# Autodesk Inventor assembly: Z Axis Motor Mount
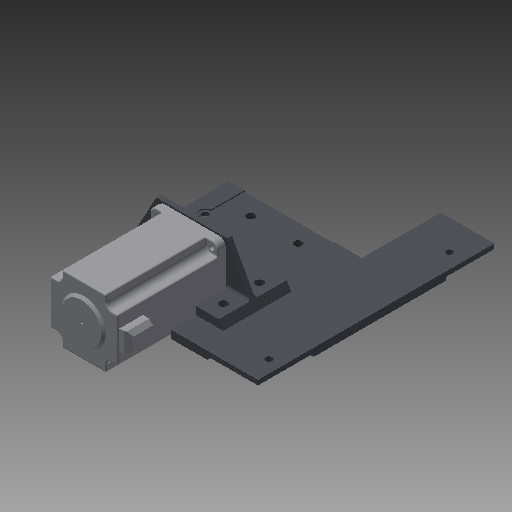
[picture p0: Inventor's stored thumbnail of the model, 512x512]
Saved by Autodesk Inventor 2018 (Build 220112000, 112)
## iProperties
Created: 2018-04-10
Part Number: Z Axis Motor Mount
Document SubType Name: Assembly
Designer: M224826
Author: M224826
## Documents named in this file (4)
- C:\Users\M224826\Documents\GitHub\CNC-Lathe-CAD\CNC Lathe Project\Project Files\Z Axis Motor Mount\Z Axis Motor Mount.iam
- C:\Users\M224826\Documents\GitHub\CNC-Lathe-CAD\CNC Lathe Project\Project Files\Servo Motor\Servo Motor.iam
- C:\Users\M224826\Documents\GitHub\CNC-Lathe-CAD\CNC Lathe Project\Project Files\Z Axis Motor Mount\Motor Support Fin.ipt
- C:\Users\M224826\Documents\GitHub\CNC-Lathe-CAD\CNC Lathe Project\Project Files\Z Axis Motor Mount\SUPPORT MAIN FRAME MOTOR-BALL SCREW-REV-B.ipt
## Components (3 placed, 3 different names)
1. Servo Motor:1 [sub-assembly] — Mate:5, Mate:6, Mate:7
2. Motor Support Fin:1 — Mate:2, Mate:3, Mate:4, Mate:5, Mate:6, Mate:7
3. SUPPORT MAIN FRAME MOTOR-BALL SCREW-REV-B:1 — Mate:1, Flush:1, Flush:2, Mate:2, Mate:3, Mate:4
## Relationships (9: Mate 7, Flush 2)
- Mate:1: SUPPORT MAIN FRAME MOTOR-BALL SCREW-REV-B:1
- Flush:1: SUPPORT MAIN FRAME MOTOR-BALL SCREW-REV-B:1
- Flush:2: SUPPORT MAIN FRAME MOTOR-BALL SCREW-REV-B:1
- Mate:2: Motor Support Fin:1 ↔ SUPPORT MAIN FRAME MOTOR-BALL SCREW-REV-B:1
- Mate:3: Motor Support Fin:1 ↔ SUPPORT MAIN FRAME MOTOR-BALL SCREW-REV-B:1
- Mate:4: Motor Support Fin:1 ↔ SUPPORT MAIN FRAME MOTOR-BALL SCREW-REV-B:1
- Mate:5: Servo Motor:1 ↔ Motor Support Fin:1
- Mate:6: Servo Motor:1 ↔ Motor Support Fin:1
- Mate:7: Servo Motor:1 ↔ Motor Support Fin:1
